# Autodesk Inventor assembly: 동작
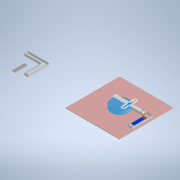
[picture p0: Inventor's stored thumbnail of the model, 180x180]
Saved by Autodesk Inventor 2022 (Build 260153000, 153)
## iProperties
Created: 2022-10-28
Part Number: 동작
Document SubType Name: Assembly
Designer: whdls
Author: whdls
## Documents named in this file (7)
- C:\Users\whdls\Desktop\대학\동아리\인벤터\스위치\동작.iam
- C:\Users\whdls\Desktop\대학\동아리\인벤터\스위치\원.ipt
- C:\Users\whdls\Desktop\대학\동아리\인벤터\스위치\축.ipt
- C:\Users\whdls\Desktop\대학\동아리\인벤터\스위치\축 케이스.ipt
- C:\Users\whdls\Desktop\대학\동아리\인벤터\스위치\수직축.ipt
- C:\Users\whdls\Desktop\대학\동아리\인벤터\스위치\배경.ipt
- C:\Users\whdls\Desktop\대학\동아리\인벤터\스위치\슬롯.ipt
## Components (8 placed, 6 different names)
1. 원:1 — 플러쉬:1, 접선:1, 메이트:3, 메이트:4
2. 축:1 — 플러쉬:1, 접선:1, 메이트:1, 플러쉬:2, 플러쉬:3, 플러쉬:6, 메이트:5
3. 축 케이스:1
4. 수직축:1 — 메이트:2, 플러쉬:2, 플러쉬:4, 메이트:6
5. 축 케이스:2 — 메이트:1, 메이트:2, 플러쉬:3, 플러쉬:4, 플러쉬:5
6. 수직축:2
7. 배경:1 — 메이트:3, 메이트:4, 플러쉬:5
8. 슬롯:1 — 플러쉬:6, 메이트:5, 메이트:6
## Relationships (13: Flush 6, Mate 6, Tangent 1)
- 플러쉬:1 [Flush]: 원:1 ↔ 축:1
- 접선:1 [Tangent]: 원:1 ↔ 축:1
- 메이트:1 [Mate]: 축:1 ↔ 축 케이스:2
- 메이트:2 [Mate]: 수직축:1 ↔ 축 케이스:2
- 플러쉬:2 [Flush]: 축:1 ↔ 수직축:1
- 플러쉬:3 [Flush]: 축:1 ↔ 축 케이스:2
- 플러쉬:4 [Flush]: 수직축:1 ↔ 축 케이스:2
- 메이트:3 [Mate]: 원:1 ↔ 배경:1
- 메이트:4 [Mate]: 원:1 ↔ 배경:1
- 플러쉬:5 [Flush]: 축 케이스:2 ↔ 배경:1
- 플러쉬:6 [Flush]: 축:1 ↔ 슬롯:1
- 메이트:5 [Mate]: 축:1 ↔ 슬롯:1
- 메이트:6 [Mate]: 수직축:1 ↔ 슬롯:1
